# Autodesk Inventor assembly: 100-10-FRAME-CHASSIS-ASM-01
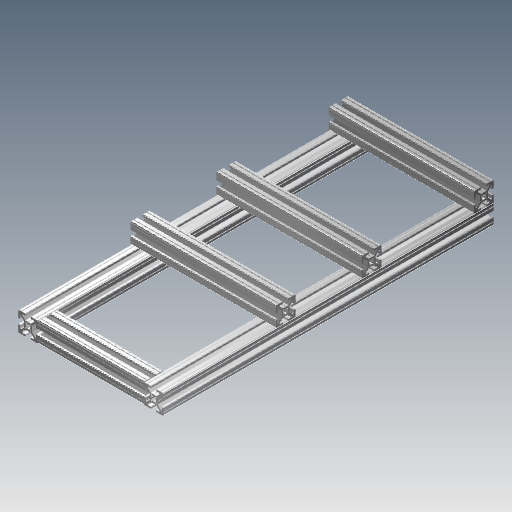
[picture p0: Inventor's stored thumbnail of the model, 512x512]
Saved by Autodesk Inventor 2018.2 (Build 222227000, 227)
## iProperties
Manager: feesmrt
Company: FRANC0R
Created: 2017-12-16
Part Number: 100-10-FRAME-CHASSIS-ASM-01
Material: Generisch
Document SubType Name: Assembly
Designer: feesmrt
Project: Rescue Robot
Cost Center: -
Description: Baseframe ASM
Engineer: feesmrt
Authority: feesmrt
Stock Number: 100-10-FRAME-CHASSIS-ASM-01
Author: feesmrt
Title: Baseframe ASM
Subject: Rescue Robot
Revision Number: 1
## Documents named in this file (6)
- D:\Programmierung\FRANC0R\CAD\02-Rocker-Bogie-Robot\100-CHASSIS\10-FRAME\100-10-FRAME-CHASSIS-ASM-01.iam
- D:\Programmierung\FRANC0R\CAD\02-Rocker-Bogie-Robot\100-CHASSIS\10-FRAME\100-10-FRAME-PROFILE-LENGTH-01.ipt
- D:\Programmierung\FRANC0R\CAD\02-Rocker-Bogie-Robot\100-CHASSIS\10-FRAME\100-10-FRAME-PROFILE-WIDTH-01.ipt
- D:\Programmierung\FRANC0R\CAD\02-Rocker-Bogie-Robot\100-CHASSIS\10-FRAME\100-10-FRAME-PROFILE-WIDTH-02.ipt
- D:\Programmierung\FRANC0R\CAD\02-Rocker-Bogie-Robot\100-CHASSIS\10-FRAME\100-10-FRAME-PROFILE-ROCKER-CONNECTOR.ipt
- D:\Programmierung\FRANC0R\CAD\02-Rocker-Bogie-Robot\100-CHASSIS\Chassis-Dimensions.xlsx
## Components (6 placed, 4 different names)
1. 100-10-FRAME-PROFILE-LENGTH-01:1 — Passend:1, Passend:4, Passend:6
2. 100-10-FRAME-PROFILE-LENGTH-01:2 — Passend:2, Passend:3, Passend:5
3. 100-10-FRAME-PROFILE-WIDTH-01:2 — Passend:10, Passend:11, Passend:12
4. 100-10-FRAME-PROFILE-WIDTH-02:1 — Passend:13, Passend:14, Fluchtend:1
5. 100-10-FRAME-PROFILE-ROCKER-CONNECTOR:1 — Passend:15, Passend:17, Fluchtend:3
6. 100-10-FRAME-PROFILE-ROCKER-CONNECTOR:2 — Passend:16, Passend:18, Fluchtend:2
## Relationships (18: Mate 15, Flush 3)
- Passend:1 [Mate]: 100-10-FRAME-PROFILE-LENGTH-01:1
- Passend:2 [Mate]: 100-10-FRAME-PROFILE-LENGTH-01:2
- Passend:3 [Mate]: 100-10-FRAME-PROFILE-LENGTH-01:2
- Passend:4 [Mate]: 100-10-FRAME-PROFILE-LENGTH-01:1
- Passend:5 [Mate] (-95 mm): 100-10-FRAME-PROFILE-LENGTH-01:2
- Passend:6 [Mate] (95 mm): 100-10-FRAME-PROFILE-LENGTH-01:1
- Passend:10 [Mate]: 100-10-FRAME-PROFILE-WIDTH-01:2
- Passend:11 [Mate]: 100-10-FRAME-PROFILE-WIDTH-01:2
- Passend:12 [Mate] (-235 mm): 100-10-FRAME-PROFILE-WIDTH-01:2
- Passend:13 [Mate] (30 mm): 100-10-FRAME-PROFILE-WIDTH-02:1
- Passend:14 [Mate]: 100-10-FRAME-PROFILE-WIDTH-02:1
- Fluchtend:1 [Flush] (235 mm): 100-10-FRAME-PROFILE-WIDTH-02:1
- Passend:15 [Mate] (30 mm): 100-10-FRAME-PROFILE-ROCKER-CONNECTOR:1
- Passend:16 [Mate] (30 mm): 100-10-FRAME-PROFILE-ROCKER-CONNECTOR:2
- Passend:17 [Mate]: 100-10-FRAME-PROFILE-ROCKER-CONNECTOR:1
- Passend:18 [Mate]: 100-10-FRAME-PROFILE-ROCKER-CONNECTOR:2
- Fluchtend:2 [Flush] (65 mm): 100-10-FRAME-PROFILE-ROCKER-CONNECTOR:2
- Fluchtend:3 [Flush] (-65 mm): 100-10-FRAME-PROFILE-ROCKER-CONNECTOR:1
## Named parameters: Chassis_Length = 500 mm, Chassis_Width = 220 mm, Chassis_Frame_Size = 30 mm, Rocker_Bearing_Size = 100 mm, Rocker_Screw_Distance = 32.5 mm
